# Autodesk Inventor assembly: Rear Lead Screw Idler
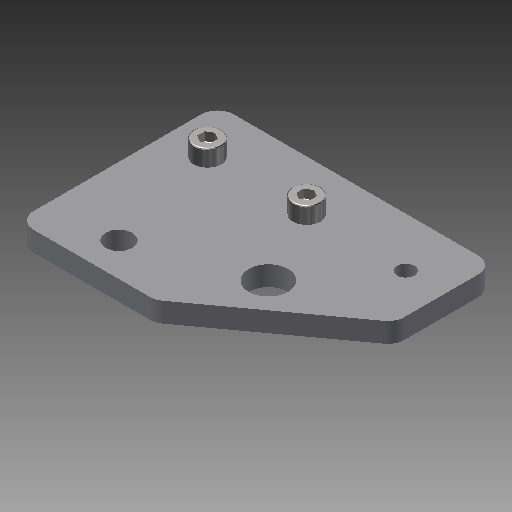
[picture p0: Inventor's stored thumbnail of the model, 512x512]
Saved by Autodesk Inventor 2017 (Build 210142000, 142)
## iProperties
Created: 2016-08-02
Part Number: Rear Lead Screw Idler
Document SubType Name: Assembly
Designer: User
Author: User
## Documents named in this file (5)
- C:\All INVENTOR\SL-Inventor\SL-Beast 3D Printer\Rear Lead Screw Idler.iam
- C:\All INVENTOR\SL-Inventor\SL-Beast 3D Printer\RearZHolder.ipt
- C:\All INVENTOR\SL-Inventor\SL-Beast 3D Printer\en-US\ANSI B18.3.1M(6)\ANSI B18.3.1M - M5x0.8 x 12(1).ipt
- C:\All INVENTOR\SL-Inventor\SL-Beast 3D Printer\M5 Tee Nut-Generic_MIR.ipt
- C:\All INVENTOR\SL-Inventor\SL-Beast 3D Printer\M5 Tee Nut-Generic_MIR_CPY1.ipt
## Components (5 placed, 4 different names)
1. RearZHolder:1
2. Forged Socket Head Cap Screw - Metric M5x0.8 x 12:1
3. Forged Socket Head Cap Screw - Metric M5x0.8 x 12:2
4. M5 Tee Nut-Generic_MIR:1
5. M5 Tee Nut-Generic_MIR_CPY1:1
## Relationships (5: Insert 2, Mate 2, Flush 1)
- [Insert]: RearZHolder:1 ↔ Forged Socket Head Cap Screw - Metric M5x0.8 x 12:1
- [Insert]: RearZHolder:1 ↔ Forged Socket Head Cap Screw - Metric M5x0.8 x 12:2
- [Mate]: Forged Socket Head Cap Screw - Metric M5x0.8 x 12:1 ↔ M5 Tee Nut-Generic_MIR_CPY1:1
- [Mate]: Forged Socket Head Cap Screw - Metric M5x0.8 x 12:2 ↔ M5 Tee Nut-Generic_MIR:1
- [Flush]: M5 Tee Nut-Generic_MIR:1 ↔ M5 Tee Nut-Generic_MIR_CPY1:1
